# Autodesk Inventor assembly: Ensamblaje_Mecanico
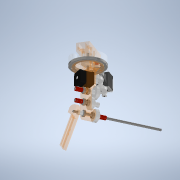
[picture p0: Inventor's stored thumbnail of the model, 180x180]
Saved by Autodesk Inventor 2021 (Build 250183000, 183)
## iProperties
Created: 2021-04-04
Part Number: Ensamblaje_Mecanico
Document SubType Name: Assembly
Designer: jorge
Author: jorge
## Documents named in this file (20)
- D:\Documentos\Inventor\Telescopio\Piezas Mecanicas\Ensamblaje_Mecanico.iam
- D:\Documentos\Inventor\Telescopio\Reduccion_Theta_3_reducciones_1.ipt
- D:\Documentos\Inventor\Telescopio\Union_fija_lazy_susan_2_1.ipt
- D:\Documentos\Inventor\Telescopio\Union_Tripode.ipt
- D:\Documentos\Inventor\Telescopio\Piezas Mecanicas\Cojinete_608zz.ipt
- D:\Documentos\Inventor\Telescopio\Piezas Mecanicas\lazy_susan.ipt
- D:\Documentos\Inventor\Telescopio\Union_rotatoria_lazy_susan.ipt
- D:\Documentos\Inventor\Telescopio\Piezas Mecanicas\Nema17.ipt
- D:\Documentos\Inventor\Telescopio\Piezas Mecanicas\chumacera.ipt
- D:\Documentos\Inventor\Telescopio\Piezas Mecanicas\Arandela.ipt
- D:\Documentos\Inventor\Telescopio\Piezas Mecanicas\Acople.ipt
- D:\Documentos\Inventor\Telescopio\Piezas Mecanicas\Gt2_20.ipt
- D:\Documentos\Inventor\Telescopio\Piezas Mecanicas\Gt2_60.ipt
- D:\Documentos\Inventor\Telescopio\Piezas Mecanicas\Gt2_20_5.ipt
- D:\Documentos\Inventor\Telescopio\Piezas Mecanicas\inox_84mm.ipt
- D:\Documentos\Inventor\Telescopio\Union_Telescopio.ipt
- D:\Documentos\Inventor\Telescopio\Piezas Mecanicas\inox_300mm.ipt
- D:\Documentos\Inventor\Telescopio\Piezas Mecanicas\inox_63mm.ipt
- D:\Documentos\Inventor\Telescopio\Piezas Mecanicas\inox_80mm.ipt
- D:\Documentos\Inventor\Telescopio\Piezas Mecanicas\inox_89mm.ipt
## Components (54 placed, 19 different names)
1. Reduccion_Theta_3_reducciones_1:1 — Mate:16, Flush:1, Mate:17, Mate:18, Mate:19, Mate:20, Mate:21, Mate:22, Mate:23, Mate:24, Mate:25, Mate:26, Mate:27, Mate:28, Mate:29, Mate:30, Mate:31, Mate:69
2. Union_fija_lazy_susan_2_1:1 — Mate:1, Mate:2, Mate:3, Mate:4, Mate:5, Mate:6, Mate:7, Mate:8, Mate:9, Mate:10, Mate:11, Mate:12, Mate:13, Mate:14, Mate:32, Mate:33, Mate:34, Mate:35, Mate:36, Mate:37, Mate:38
3. Union_Tripode:1 — Mate:1, Mate:2, Mate:5, Mate:92
4. Cojinete_608zz:1 — Mate:3, Mate:4, Mate:91
5. Cojinete_608zz:2 — Mate:10, Mate:11, Mate:56, Mate:57
6. Cojinete_608zz:3 — Mate:8, Mate:9, Mate:48, Mate:49
7. Cojinete_608zz:4 — Mate:6, Mate:7, Mate:39, Mate:46, Mate:47, Mate:96
8. lazy_susan:1 — Mate:12, Mate:13, Mate:14, Mate:15, Mate:94
9. Union_rotatoria_lazy_susan:1 — Mate:15, Mate:16, Flush:1, Mate:80, Mate:81, Mate:94
10. Cojinete_608zz:5 — Mate:17, Mate:18, Mate:44, Mate:45
11. Cojinete_608zz:6 — Mate:19, Mate:20, Mate:42, Mate:43, Mate:73
12. Cojinete_608zz:7 — Mate:25, Mate:26, Mate:52, Mate:53
13. Cojinete_608zz:8 — Mate:21, Mate:22, Mate:40, Mate:41
14. Cojinete_608zz:9 — Mate:27, Mate:28, Mate:54, Mate:55, Mate:63, Mate:77
15. Cojinete_608zz:10 — Mate:23, Mate:24, Mate:50, Mate:51, Mate:86
16. Nema17:1 — Mate:29, Mate:30, Mate:31, Mate:82, Flush:2
17. Nema17:2 — Mate:32, Mate:33, Mate:34, Mate:103, Mate:116
18. chumacera:1 — Mate:35, Mate:36, Mate:37
19. Cojinete_608zz:11 — Mate:38, Mate:39, Mate:58, Mate:59
20. Arandela:1 — Mate:46, Mate:47, Mate:95
21. Arandela:2 — Mate:42, Mate:43, Mate:72
22. Arandela:3 — Mate:40, Mate:41, Mate:76
23. Arandela:4 — Mate:44, Mate:45, Mate:68
24. Arandela:5 — Mate:48, Mate:49, Mate:112
25. Arandela:6 — Mate:50, Mate:51, Mate:85
26. Arandela:7 — Mate:52, Mate:53, Mate:60, Mate:61
27. Arandela:8 — Mate:54, Mate:55, Mate:62
28. Arandela:9 — Mate:56, Mate:57, Mate:66, Mate:67
29. Arandela:10 — Mate:58, Mate:59, Mate:64, Mate:65
30. Acople:1 — Mate:60, Mate:61, Mate:84
31. Acople:2 — Mate:62, Mate:63, Mate:83
32. Acople:3 — Mate:64, Mate:65, Mate:107, Flush:7
33. Acople:4 — Mate:66, Mate:67, Mate:110, Mate:111
34. Gt2_20:1 — Mate:74, Mate:75, Flush:4
35. Gt2_60:1 — Mate:68, Mate:69, Mate:70, Mate:71
36. Acople:5 — Mate:70, Mate:71
37. Gt2_60:2 — Mate:72, Mate:73, Mate:74, Mate:75
38. Gt2_20:2 — Mate:76, Mate:77, Mate:78, Mate:79
39. Gt2_60:3 — Mate:78, Mate:79, Flush:3
40. Gt2_60:4 — Mate:80, Mate:81, Mate:93
41. Gt2_20_5:1 — Mate:82, Flush:2
42. inox_84mm:1 — Mate:83, Flush:3
43. inox_84mm:2 — Mate:84, Flush:4
44. Gt2_20:3 — Mate:85, Mate:86, Mate:87, Mate:88
45. Union_Telescopio:1 — Mate:87, Mate:88, Mate:89, Mate:90
46. inox_300mm:1 — Mate:89, Mate:90
47. inox_63mm:1 — Mate:91, Mate:92, Mate:93
48. Gt2_20:4 — Mate:95, Mate:96, Mate:109
49. Gt2_60:5 — Mate:108, Mate:109
50. Gt2_20:5 — Mate:112, Mate:113, Mate:114
51. Gt2_60:6 — Mate:114, Mate:115
52. Gt2_20_5:2 — Mate:103, Mate:116
53. inox_80mm:1 — Mate:107, Flush:7, Mate:108
54. inox_89mm:1 — Mate:110, Mate:111, Mate:113, Mate:115
## Relationships (112: Mate 107, Flush 5)
- Mate:1: Union_fija_lazy_susan_2_1:1 ↔ Union_Tripode:1
- Mate:2: Union_fija_lazy_susan_2_1:1 ↔ Union_Tripode:1
- Mate:3: Union_fija_lazy_susan_2_1:1 ↔ Cojinete_608zz:1
- Mate:4: Union_fija_lazy_susan_2_1:1 ↔ Cojinete_608zz:1
- Mate:5: Union_fija_lazy_susan_2_1:1 ↔ Union_Tripode:1
- Mate:6: Union_fija_lazy_susan_2_1:1 ↔ Cojinete_608zz:4
- Mate:7: Union_fija_lazy_susan_2_1:1 ↔ Cojinete_608zz:4
- Mate:8: Union_fija_lazy_susan_2_1:1 ↔ Cojinete_608zz:3
- Mate:9: Union_fija_lazy_susan_2_1:1 ↔ Cojinete_608zz:3
- Mate:10: Union_fija_lazy_susan_2_1:1 ↔ Cojinete_608zz:2
- Mate:11: Union_fija_lazy_susan_2_1:1 ↔ Cojinete_608zz:2
- Mate:12: Union_fija_lazy_susan_2_1:1 ↔ lazy_susan:1
- Mate:13: Union_fija_lazy_susan_2_1:1 ↔ lazy_susan:1
- Mate:14: Union_fija_lazy_susan_2_1:1 ↔ lazy_susan:1
- Mate:15: lazy_susan:1 ↔ Union_rotatoria_lazy_susan:1
- Mate:16: Reduccion_Theta_3_reducciones_1:1 ↔ Union_rotatoria_lazy_susan:1
- Flush:1: Reduccion_Theta_3_reducciones_1:1 ↔ Union_rotatoria_lazy_susan:1
- Mate:17: Reduccion_Theta_3_reducciones_1:1 ↔ Cojinete_608zz:5
- Mate:18: Reduccion_Theta_3_reducciones_1:1 ↔ Cojinete_608zz:5
- Mate:19: Reduccion_Theta_3_reducciones_1:1 ↔ Cojinete_608zz:6
- Mate:20: Reduccion_Theta_3_reducciones_1:1 ↔ Cojinete_608zz:6
- Mate:21: Reduccion_Theta_3_reducciones_1:1 ↔ Cojinete_608zz:8
- Mate:22: Reduccion_Theta_3_reducciones_1:1 ↔ Cojinete_608zz:8
- Mate:23: Reduccion_Theta_3_reducciones_1:1 ↔ Cojinete_608zz:10
- Mate:24: Reduccion_Theta_3_reducciones_1:1 ↔ Cojinete_608zz:10
- Mate:25: Reduccion_Theta_3_reducciones_1:1 ↔ Cojinete_608zz:7
- Mate:26: Reduccion_Theta_3_reducciones_1:1 ↔ Cojinete_608zz:7
- Mate:27: Reduccion_Theta_3_reducciones_1:1 ↔ Cojinete_608zz:9
- Mate:28: Reduccion_Theta_3_reducciones_1:1 ↔ Cojinete_608zz:9
- Mate:29: Reduccion_Theta_3_reducciones_1:1 ↔ Nema17:1
- Mate:30: Reduccion_Theta_3_reducciones_1:1 ↔ Nema17:1
- Mate:31: Reduccion_Theta_3_reducciones_1:1 ↔ Nema17:1
- Mate:32: Union_fija_lazy_susan_2_1:1 ↔ Nema17:2
- Mate:33: Union_fija_lazy_susan_2_1:1 ↔ Nema17:2
- Mate:34: Union_fija_lazy_susan_2_1:1 ↔ Nema17:2
- Mate:35: Union_fija_lazy_susan_2_1:1 ↔ chumacera:1
- Mate:36: Union_fija_lazy_susan_2_1:1 ↔ chumacera:1
- Mate:37: Union_fija_lazy_susan_2_1:1 ↔ chumacera:1
- Mate:38: Union_fija_lazy_susan_2_1:1 ↔ Cojinete_608zz:11
- Mate:39: Cojinete_608zz:4 ↔ Cojinete_608zz:11
- Mate:40: Cojinete_608zz:8 ↔ Arandela:3
- Mate:41: Cojinete_608zz:8 ↔ Arandela:3
- Mate:42: Cojinete_608zz:6 ↔ Arandela:2
- Mate:43: Cojinete_608zz:6 ↔ Arandela:2
- Mate:44: Cojinete_608zz:5 ↔ Arandela:4
- Mate:45: Cojinete_608zz:5 ↔ Arandela:4
- Mate:46: Cojinete_608zz:4 ↔ Arandela:1
- Mate:47: Cojinete_608zz:4 ↔ Arandela:1
- Mate:48: Cojinete_608zz:3 ↔ Arandela:5
- Mate:49: Cojinete_608zz:3 ↔ Arandela:5
- Mate:50: Cojinete_608zz:10 ↔ Arandela:6
- Mate:51: Cojinete_608zz:10 ↔ Arandela:6
- Mate:52: Cojinete_608zz:7 ↔ Arandela:7
- Mate:53: Cojinete_608zz:7 ↔ Arandela:7
- Mate:54: Cojinete_608zz:9 ↔ Arandela:8
- Mate:55: Cojinete_608zz:9 ↔ Arandela:8
- Mate:56: Cojinete_608zz:2 ↔ Arandela:9
- Mate:57: Cojinete_608zz:2 ↔ Arandela:9
- Mate:58: Cojinete_608zz:11 ↔ Arandela:10
- Mate:59: Cojinete_608zz:11 ↔ Arandela:10
- Mate:60: Arandela:7 ↔ Acople:1
- Mate:61: Arandela:7 ↔ Acople:1
- Mate:62: Arandela:8 ↔ Acople:2
- Mate:63: Cojinete_608zz:9 ↔ Acople:2
- Mate:64: Arandela:10 ↔ Acople:3
- Mate:65: Arandela:10 ↔ Acople:3
- Mate:66: Arandela:9 ↔ Acople:4
- Mate:67: Arandela:9 ↔ Acople:4
- Mate:68: Arandela:4 ↔ Gt2_60:1
- Mate:69: Reduccion_Theta_3_reducciones_1:1 ↔ Gt2_60:1
- Mate:70: Gt2_60:1 ↔ Acople:5
- Mate:71: Gt2_60:1 ↔ Acople:5
- Mate:72: Arandela:2 ↔ Gt2_60:2
- Mate:73: Cojinete_608zz:6 ↔ Gt2_60:2
- Mate:74: Gt2_20:1 ↔ Gt2_60:2
- Mate:75: Gt2_20:1 ↔ Gt2_60:2
- Mate:76: Arandela:3 ↔ Gt2_20:2
- Mate:77: Cojinete_608zz:9 ↔ Gt2_20:2
- Mate:78: Gt2_20:2 ↔ Gt2_60:3
- Mate:79: Gt2_20:2 ↔ Gt2_60:3
- Mate:80: Union_rotatoria_lazy_susan:1 ↔ Gt2_60:4
- Mate:81: Union_rotatoria_lazy_susan:1 ↔ Gt2_60:4
- Mate:82: Nema17:1 ↔ Gt2_20_5:1
- Flush:2 (4 mm): Nema17:1 ↔ Gt2_20_5:1
- Mate:83: Acople:2 ↔ inox_84mm:1
- Flush:3 (-2 mm): Gt2_60:3 ↔ inox_84mm:1
- Mate:84: Acople:1 ↔ inox_84mm:2
- Flush:4 (-2 mm): Gt2_20:1 ↔ inox_84mm:2
- Mate:85: Arandela:6 ↔ Gt2_20:3
- Mate:86: Cojinete_608zz:10 ↔ Gt2_20:3
- Mate:87: Gt2_20:3 ↔ Union_Telescopio:1
- Mate:88: Gt2_20:3 ↔ Union_Telescopio:1
- Mate:89: Union_Telescopio:1 ↔ inox_300mm:1
- Mate:90 (-16 mm): Union_Telescopio:1 ↔ inox_300mm:1
- Mate:91: Cojinete_608zz:1 ↔ inox_63mm:1
- Mate:92: Union_Tripode:1 ↔ inox_63mm:1
- Mate:93: Gt2_60:4 ↔ inox_63mm:1
- Mate:94: lazy_susan:1 ↔ Union_rotatoria_lazy_susan:1
- Mate:95: Arandela:1 ↔ Gt2_20:4
- Mate:96: Cojinete_608zz:4 ↔ Gt2_20:4
- Mate:103: Nema17:2 ↔ Gt2_20_5:2
- Mate:107: Acople:3 ↔ inox_80mm:1
- Flush:7 (-2 mm): Acople:3 ↔ inox_80mm:1
- Mate:108: Gt2_60:5 ↔ inox_80mm:1
- Mate:109: Gt2_20:4 ↔ Gt2_60:5
- Mate:110: Acople:4 ↔ inox_89mm:1
- Mate:111 (2 mm): Acople:4 ↔ inox_89mm:1
- Mate:112: Arandela:5 ↔ Gt2_20:5
- Mate:113: Gt2_20:5 ↔ inox_89mm:1
- Mate:114: Gt2_20:5 ↔ Gt2_60:6
- Mate:115: Gt2_60:6 ↔ inox_89mm:1
- Mate:116 (2 mm): Nema17:2 ↔ Gt2_20_5:2
